# Autodesk Inventor assembly: SERVO
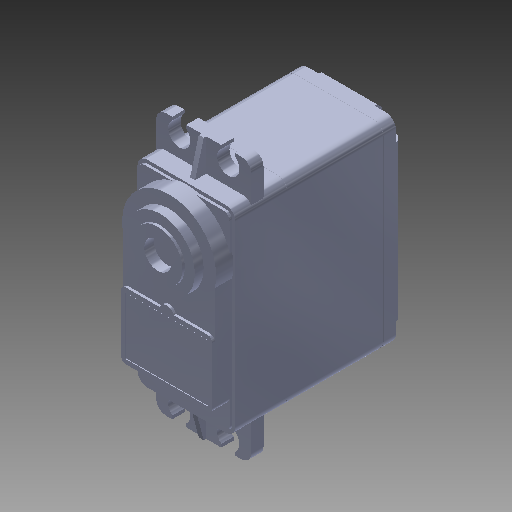
[picture p0: Inventor's stored thumbnail of the model, 512x512]
Saved by Autodesk Inventor 2019 (Build 230136000, 136)
## iProperties
Created: 2012-10-11
Part Number: SERVO
Document SubType Name: Assembly
Designer: Mario
Sending System: SolidWorks 2012
Last Author: Utente
Last Saved: 2014-01-18
Author: Mario
## Documents named in this file (3)
- D:\Documents\Kevin\robot\SERVOBRAZO.iam
- D:\Documents\Kevin\robot\SERVOMOTORE Hitec HS485-HB.ipt
- C:\Users\Kevin\Desktop\tesisVero\PartesRobot\Ingranaggio dentato innesto servomotore.ipt
## Components (2 placed, 2 different names)
1. SERVOMOTORE Hitec HS485-HB:1 — Insert:2
2. Ingranaggio dentato innesto servomotore:1 — Insert:2
## Relationships (1: Insert 1)
- Insert:2: SERVOMOTORE Hitec HS485-HB:1 ↔ Ingranaggio dentato innesto servomotore:1
